# Autodesk Inventor assembly: 6whalfdt_MIR
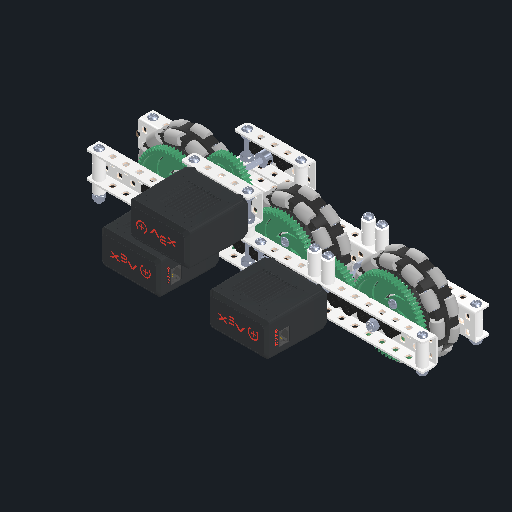
[picture p0: Inventor's stored thumbnail of the model, 512x512]
Saved by Autodesk Inventor 2024 (Build 280153000, 153)
## iProperties
Created: 2023-08-12
Part Number: 6whalfdt_MIR
Document SubType Name: Assembly
Designer: macbook
Author: macbook
## Documents named in this file (15)
- \\Mac\Home\Desktop\code\7899V-VRC-OVER-UNDER\Cad\VEX-CAD-Inventor-1.4.0\Assembly\v0.2\6whalfdt_MIR.iam
- \\Mac\Home\Desktop\code\7899V-VRC-OVER-UNDER\Cad\VEX-CAD-Inventor-1.4.0\Assembly\v0.2\wheel1_MIR.iam
- \\Mac\Home\Desktop\code\7899V-VRC-OVER-UNDER\Cad\VEX-CAD-Inventor-1.4.0\Assembly\v0.2\wheel2_MIR.iam
- \\Mac\Home\Desktop\code\7899V-VRC-OVER-UNDER\Cad\VEX-CAD-Inventor-1.4.0\Assembly\v0.2\wheel4_MIR.iam
- \\Mac\Home\Desktop\code\7899V-VRC-OVER-UNDER\Cad\VEX-CAD-Inventor-1.4.0\Structure\C Channel\Aluminum 1x2x1\Alu C 1x2x1x25_MIR1.ipt
- \\Mac\Home\Desktop\code\7899V-VRC-OVER-UNDER\Cad\VEX-CAD-Inventor-1.4.0\Motion\Spacers\Spacer Nylon .313 OD\NSpacer .313 OD x .375.ipt
- \\Mac\Home\Desktop\code\7899V-VRC-OVER-UNDER\Cad\VEX-CAD-Inventor-1.4.0\Motion\Spacers\Spacer Nylon .313 OD.ipt
- \\Mac\Home\Desktop\code\7899V-VRC-OVER-UNDER\Cad\VEX-CAD-Inventor-1.4.0\Motion\Spacers\box.iam
- \\Mac\Home\Desktop\code\7899V-VRC-OVER-UNDER\Cad\VEX-CAD-Inventor-1.4.0\Structure\Hardware\Screw Steel - Star\SScrew Star Smooth 1.750.ipt
- \\Mac\Home\Desktop\code\7899V-VRC-OVER-UNDER\Cad\VEX-CAD-Inventor-1.4.0\Structure\Hardware\Screw Steel - Star.ipt
- \\Mac\Home\Desktop\code\7899V-VRC-OVER-UNDER\Cad\VEX-CAD-Inventor-1.4.0\Structure\Hardware\Nut Nylock_MIR1.ipt
- \\Mac\Home\Desktop\code\7899V-VRC-OVER-UNDER\Cad\VEX-CAD-Inventor-1.4.0\Structure\Hardware\Screw Steel - Star\SScrew Star Smooth 1.250.ipt
- \\Mac\Home\Desktop\code\7899V-VRC-OVER-UNDER\Cad\VEX-CAD-Inventor-1.4.0\Structure\Hardware\Nut Keps_MIR.ipt
- \\Mac\Home\Desktop\code\7899V-VRC-OVER-UNDER\Cad\VEX-CAD-Inventor-1.4.0\Structure\Hardware\Nut Thin Nylock_MIR1.ipt
- \\Mac\Home\Desktop\code\7899V-VRC-OVER-UNDER\Cad\VEX-CAD-Inventor-1.4.0\Structure\Hardware\Screw Steel - Star\SScrew Star Smooth 1.000.ipt
## Components (45 placed, 12 different names)
1. wheel1_MIR:1 [sub-assembly] — Insert:10, Insert:9
2. wheel1_MIR:2 [sub-assembly] — Insert:6, Insert:5
3. wheel2_MIR:1 [sub-assembly] — Insert:4, Insert:3
4. wheel1_MIR:3 [sub-assembly] — Insert:2, Insert:1
5. wheel4_MIR:1 [sub-assembly] — Insert:14, Insert:13
6. wheel2_MIR:2 [sub-assembly] — Insert:8, Insert:7
7. Alu C 1x2x1x25_MIR1:1 — Insert:14, Insert:13, Insert:10, Insert:9, Insert:6, Insert:5, Insert:4, Insert:3, Insert:2, Insert:1, Insert:12, Insert:11, Insert:8, Insert:7, Insert:16, Insert:18, Insert:19, Insert:23, Insert:25, Insert:27, Insert:35, Insert:37, Insert:41, Insert:40, Insert:42, Insert:43
8. Alu C 1x2x1x25_MIR1:2 — Insert:12, Insert:11, Insert:15, Insert:17, Insert:21, Insert:24, Insert:26, Insert:28, Insert:29, Insert:31, Insert:30, Insert:33, Insert:32, Insert:45, Insert:44, Insert:51, Insert:50
9. NSpacer .313 OD x .375:1 — Insert:16, Insert:20
10. NSpacer .313 OD x .375:2 — Insert:15, Insert:22
11. box:1 [sub-assembly] — Insert:17
12. box:2 [sub-assembly] — Insert:18
13. SScrew Star Smooth 1.750:1 — Insert:19
14. SScrew Star Smooth 1.750:2 — Insert:21
15. Nut Nylock_MIR1:1 — Insert:20
16. Nut Nylock_MIR1:2 — Insert:22
17. box:3 [sub-assembly] — Insert:23
18. box:4 [sub-assembly] — Insert:24
19. SScrew Star Smooth 1.250:3 — Insert:25
20. SScrew Star Smooth 1.250:4 — Insert:26
21. Nut Nylock_MIR1:3 — Insert:27
22. Nut Nylock_MIR1:4 — Insert:28
23. SScrew Star Smooth 1.250:5 — Insert:29
24. Nut Keps_MIR:1 — Insert:31
25. Nut Keps_MIR:2 — Insert:30
26. Nut Thin Nylock_MIR1:1 — Insert:33
27. Nut Thin Nylock_MIR1:2 — Insert:32
28. NSpacer .313 OD x .375:3 — Insert:34, Insert:38
29. NSpacer .313 OD x .375:4 — Insert:35, Insert:34
30. NSpacer .313 OD x .375:5 — Insert:37, Insert:36
31. NSpacer .313 OD x .375:6 — Insert:36, Insert:39
32. SScrew Star Smooth 1.750:6 — Insert:38
33. SScrew Star Smooth 1.750:7 — Insert:39
34. Nut Keps_MIR:3 — Insert:41
35. Nut Keps_MIR:4 — Insert:40
36. Nut Keps_MIR:5 — Insert:42
37. Nut Keps_MIR:6 — Insert:43
38. Nut Nylock_MIR1:5 — Insert:45
39. Nut Nylock_MIR1:6 — Insert:44
40. NSpacer .313 OD x .375:7 — Insert:46, Insert:47
41. NSpacer .313 OD x .375:8 — Insert:51, Insert:46
42. SScrew Star Smooth 1.000:8 — Insert:47
43. NSpacer .313 OD x .375:9 — Insert:48, Insert:49
44. NSpacer .313 OD x .375:10 — Insert:50, Insert:48
45. SScrew Star Smooth 1.000:9 — Insert:49
## Relationships (51: Insert 51)
- Insert:14: wheel4_MIR:1 ↔ Alu C 1x2x1x25_MIR1:1
- Insert:13: wheel4_MIR:1 ↔ Alu C 1x2x1x25_MIR1:1
- Insert:10: wheel1_MIR:1 ↔ Alu C 1x2x1x25_MIR1:1
- Insert:9: wheel1_MIR:1 ↔ Alu C 1x2x1x25_MIR1:1
- Insert:6: wheel1_MIR:2 ↔ Alu C 1x2x1x25_MIR1:1
- Insert:5: wheel1_MIR:2 ↔ Alu C 1x2x1x25_MIR1:1
- Insert:4: wheel2_MIR:1 ↔ Alu C 1x2x1x25_MIR1:1
- Insert:3: wheel2_MIR:1 ↔ Alu C 1x2x1x25_MIR1:1
- Insert:2: wheel1_MIR:3 ↔ Alu C 1x2x1x25_MIR1:1
- Insert:1: wheel1_MIR:3 ↔ Alu C 1x2x1x25_MIR1:1
- Insert:12 (34.925 mm): Alu C 1x2x1x25_MIR1:1 ↔ Alu C 1x2x1x25_MIR1:2
- Insert:11 (34.925 mm): Alu C 1x2x1x25_MIR1:1 ↔ Alu C 1x2x1x25_MIR1:2
- Insert:8: wheel2_MIR:2 ↔ Alu C 1x2x1x25_MIR1:1
- Insert:7: wheel2_MIR:2 ↔ Alu C 1x2x1x25_MIR1:1
- Insert:16: Alu C 1x2x1x25_MIR1:1 ↔ NSpacer .313 OD x .375:1
- Insert:15: Alu C 1x2x1x25_MIR1:2 ↔ NSpacer .313 OD x .375:2
- Insert:17: Alu C 1x2x1x25_MIR1:2 ↔ box:1
- Insert:18: Alu C 1x2x1x25_MIR1:1 ↔ box:2
- Insert:19: Alu C 1x2x1x25_MIR1:1 ↔ SScrew Star Smooth 1.750:1
- Insert:21: Alu C 1x2x1x25_MIR1:2 ↔ SScrew Star Smooth 1.750:2
- Insert:20 (1.5875 mm): NSpacer .313 OD x .375:1 ↔ Nut Nylock_MIR1:1
- Insert:22 (1.5875 mm): NSpacer .313 OD x .375:2 ↔ Nut Nylock_MIR1:2
- Insert:23: Alu C 1x2x1x25_MIR1:1 ↔ box:3
- Insert:24: Alu C 1x2x1x25_MIR1:2 ↔ box:4
- Insert:25: Alu C 1x2x1x25_MIR1:1 ↔ SScrew Star Smooth 1.250:3
- Insert:26: Alu C 1x2x1x25_MIR1:2 ↔ SScrew Star Smooth 1.250:4
- Insert:27: Alu C 1x2x1x25_MIR1:1 ↔ Nut Nylock_MIR1:3
- Insert:28: Alu C 1x2x1x25_MIR1:2 ↔ Nut Nylock_MIR1:4
- Insert:29: Alu C 1x2x1x25_MIR1:2 ↔ SScrew Star Smooth 1.250:5
- Insert:31: Alu C 1x2x1x25_MIR1:2 ↔ Nut Keps_MIR:1
- Insert:30: Alu C 1x2x1x25_MIR1:2 ↔ Nut Keps_MIR:2
- Insert:33 (1.5875 mm): Alu C 1x2x1x25_MIR1:2 ↔ Nut Thin Nylock_MIR1:1
- Insert:32 (1.5875 mm): Alu C 1x2x1x25_MIR1:2 ↔ Nut Thin Nylock_MIR1:2
- Insert:35: Alu C 1x2x1x25_MIR1:1 ↔ NSpacer .313 OD x .375:4
- Insert:34: NSpacer .313 OD x .375:3 ↔ NSpacer .313 OD x .375:4
- Insert:37: Alu C 1x2x1x25_MIR1:1 ↔ NSpacer .313 OD x .375:5
- Insert:36: NSpacer .313 OD x .375:5 ↔ NSpacer .313 OD x .375:6
- Insert:38 (1.5875 mm): NSpacer .313 OD x .375:3 ↔ SScrew Star Smooth 1.750:6
- Insert:39 (1.5875 mm): NSpacer .313 OD x .375:6 ↔ SScrew Star Smooth 1.750:7
- Insert:41: Alu C 1x2x1x25_MIR1:1 ↔ Nut Keps_MIR:3
- Insert:40: Alu C 1x2x1x25_MIR1:1 ↔ Nut Keps_MIR:4
- Insert:42: Alu C 1x2x1x25_MIR1:1 ↔ Nut Keps_MIR:5
- Insert:43: Alu C 1x2x1x25_MIR1:1 ↔ Nut Keps_MIR:6
- Insert:45: Alu C 1x2x1x25_MIR1:2 ↔ Nut Nylock_MIR1:5
- Insert:44: Alu C 1x2x1x25_MIR1:2 ↔ Nut Nylock_MIR1:6
- Insert:51: Alu C 1x2x1x25_MIR1:2 ↔ NSpacer .313 OD x .375:8
- Insert:46: NSpacer .313 OD x .375:7 ↔ NSpacer .313 OD x .375:8
- Insert:47 (1.5875 mm): NSpacer .313 OD x .375:7 ↔ SScrew Star Smooth 1.000:8
- Insert:50: Alu C 1x2x1x25_MIR1:2 ↔ NSpacer .313 OD x .375:10
- Insert:48: NSpacer .313 OD x .375:9 ↔ NSpacer .313 OD x .375:10
- Insert:49 (1.5875 mm): NSpacer .313 OD x .375:9 ↔ SScrew Star Smooth 1.000:9
